# Autodesk Inventor assembly: Basic Chassis
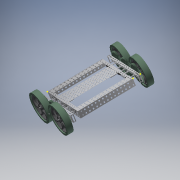
[picture p0: Inventor's stored thumbnail of the model, 180x180]
Saved by Autodesk Inventor 2018 (Build 220112000, 112)
## iProperties
Created: 2018-10-17
Part Number: Basic Chassis
Document SubType Name: Assembly
Designer: USER
Author: USER
## Documents named in this file (9)
- C:\Users\USER\Downloads\Inventor\Basic Chassis.iam
- C:\Users\USER\Downloads\Inventor\flat metal frame.ipt
- C:\Users\USER\Downloads\Inventor\Wheel.ipt
- C:\Users\USER\Downloads\Inventor\2sqr x 2sqr metal frame.ipt
- C:\Users\USER\Downloads\Inventor\1sqr x 2sqr metal frame.ipt
- C:\Users\USER\Downloads\Inventor\Axle.ipt
- C:\Users\USER\Downloads\Inventor\Gear.ipt
- C:\Users\USER\Downloads\Inventor\Plastic Fastener.ipt
- C:\Users\USER\Downloads\Inventor\Metal Fastener.ipt
## Components (34 placed, 8 different names)
1. flat metal frame:1 — Rigid:6
2. Wheel:2
3. 2sqr x 2sqr metal frame:1 — Mate:1, Mate:2, Mate:3, Mate:4, Flush:2, Flush:5
4. 2sqr x 2sqr metal frame:2 — Mate:5, Mate:6
5. 1sqr x 2sqr metal frame:1 — Mate:1, Mate:2, Mate:5, Mate:6, Flush:1, Flush:6, Rigid:6, Rigid:7, Rigid:9, Rigid:11
6. 1sqr x 2sqr metal frame:2 — Mate:3, Mate:4, Flush:3, Flush:4, Rigid:15, Rigid:16, Rigid:17
7. 1sqr x 2sqr metal frame:3 — Flush:3, Flush:4, Flush:5, Rigid:23, Rigid:24
8. 1sqr x 2sqr metal frame:4 — Flush:1, Flush:2, Flush:6, Rigid:25, Rigid:26
9. Axle:1 — Rotational:1, Rigid:8, Rigid:14
10. Axle:7 — Rotational:2, Rigid:10
11. Gear:3 — Rigid:10, Rotation:1, Rotation:2
12. Gear:6 — Rigid:8, Rotation:1
13. Plastic Fastener:2 — Rigid:7, Rotational:1
14. Plastic Fastener:6 — Rigid:9, Rotational:2
15. Plastic Fastener:7 — Rigid:11, Rotational:3
16. Axle:8 — Rotational:3, Rigid:12, Rigid:13
17. Gear:7 — Rigid:12, Rotation:2
18. Wheel:3 — Rigid:13
19. Wheel:4 — Rigid:14
20. Plastic Fastener:8 — Rigid:15, Rotational:4
21. Plastic Fastener:9 — Rigid:16, Rotational:5
22. Plastic Fastener:10 — Rigid:17, Rotational:6
23. Axle:9 — Rotational:6, Rigid:18, Rigid:22
24. Axle:10 — Rotational:4, Rigid:20, Rigid:21
25. Axle:11 — Rotational:5, Rigid:19
26. Gear:8 — Rigid:19, Rotation:3, Rotation:4
27. Gear:9 — Rigid:18, Rotation:3
28. Gear:10 — Rigid:20, Rotation:4
29. Wheel:5 — Rigid:21
30. Wheel:6 — Rigid:22
31. Metal Fastener:1 — Rigid:23
32. Metal Fastener:2 — Rigid:25
33. Metal Fastener:3 — Rigid:24
34. Metal Fastener:4 — Rigid:26
## Relationships (43: WeldJoint 21, Mate 6, Flush 6, RevoluteJoint 6, RelateRotation 4)
- Mate:1: 2sqr x 2sqr metal frame:1 ↔ 1sqr x 2sqr metal frame:1
- Mate:2: 2sqr x 2sqr metal frame:1 ↔ 1sqr x 2sqr metal frame:1
- Mate:3: 2sqr x 2sqr metal frame:1 ↔ 1sqr x 2sqr metal frame:2
- Mate:4: 2sqr x 2sqr metal frame:1 ↔ 1sqr x 2sqr metal frame:2
- Mate:5: 2sqr x 2sqr metal frame:2 ↔ 1sqr x 2sqr metal frame:1
- Mate:6: 2sqr x 2sqr metal frame:2 ↔ 1sqr x 2sqr metal frame:1
- Flush:1 (-25.4 mm): 1sqr x 2sqr metal frame:1 ↔ 1sqr x 2sqr metal frame:4
- Flush:2: 2sqr x 2sqr metal frame:1 ↔ 1sqr x 2sqr metal frame:4
- Flush:3 (-25.4 mm): 1sqr x 2sqr metal frame:2 ↔ 1sqr x 2sqr metal frame:3
- Flush:4: 1sqr x 2sqr metal frame:2 ↔ 1sqr x 2sqr metal frame:3
- Flush:5: 2sqr x 2sqr metal frame:1 ↔ 1sqr x 2sqr metal frame:3
- Flush:6: 1sqr x 2sqr metal frame:1 ↔ 1sqr x 2sqr metal frame:4
- Rigid:6 [WeldJoint]: flat metal frame:1 ↔ 1sqr x 2sqr metal frame:1
- Rigid:7 [WeldJoint]: 1sqr x 2sqr metal frame:1 ↔ Plastic Fastener:2
- Rotational:1 [RevoluteJoint] (-25 mm): Axle:1 ↔ Plastic Fastener:2
- Rigid:8 [WeldJoint] (-20 mm): Axle:1 ↔ Gear:6
- Rigid:9 [WeldJoint]: 1sqr x 2sqr metal frame:1 ↔ Plastic Fastener:6
- Rotational:2 [RevoluteJoint] (-25 mm): Axle:7 ↔ Plastic Fastener:6
- Rigid:10 [WeldJoint] (-20 mm): Axle:7 ↔ Gear:3
- Rotation:1 [RelateRotation] (1 ul): Gear:3 ↔ Gear:6
- Rigid:11 [WeldJoint]: 1sqr x 2sqr metal frame:1 ↔ Plastic Fastener:7
- Rotational:3 [RevoluteJoint] (-25 mm): Plastic Fastener:7 ↔ Axle:8
- Rigid:12 [WeldJoint] (-20 mm): Axle:8 ↔ Gear:7
- Rotation:2 [RelateRotation] (1 ul): Gear:3 ↔ Gear:7
- Rigid:13 [WeldJoint] (-15 mm): Axle:8 ↔ Wheel:3
- Rigid:14 [WeldJoint] (-15 mm): Axle:1 ↔ Wheel:4
- Rigid:15 [WeldJoint]: 1sqr x 2sqr metal frame:2 ↔ Plastic Fastener:8
- Rigid:16 [WeldJoint]: 1sqr x 2sqr metal frame:2 ↔ Plastic Fastener:9
- Rigid:17 [WeldJoint]: 1sqr x 2sqr metal frame:2 ↔ Plastic Fastener:10
- Rotational:4 [RevoluteJoint] (25 mm): Plastic Fastener:8 ↔ Axle:10
- Rotational:5 [RevoluteJoint] (-25 mm): Plastic Fastener:9 ↔ Axle:11
- Rotational:6 [RevoluteJoint] (-25 mm): Plastic Fastener:10 ↔ Axle:9
- Rigid:18 [WeldJoint] (-20 mm): Axle:9 ↔ Gear:9
- Rigid:19 [WeldJoint] (-22 mm): Axle:11 ↔ Gear:8
- Rotation:3 [RelateRotation] (1 ul): Gear:8 ↔ Gear:9
- Rigid:20 [WeldJoint] (-20 mm): Axle:10 ↔ Gear:10
- Rotation:4 [RelateRotation] (1 ul): Gear:8 ↔ Gear:10
- Rigid:21 [WeldJoint] (-15 mm): Axle:10 ↔ Wheel:5
- Rigid:22 [WeldJoint] (-15 mm): Axle:9 ↔ Wheel:6
- Rigid:23 [WeldJoint]: 1sqr x 2sqr metal frame:3 ↔ Metal Fastener:1
- Rigid:24 [WeldJoint]: 1sqr x 2sqr metal frame:3 ↔ Metal Fastener:3
- Rigid:25 [WeldJoint]: 1sqr x 2sqr metal frame:4 ↔ Metal Fastener:2
- Rigid:26 [WeldJoint]: 1sqr x 2sqr metal frame:4 ↔ Metal Fastener:4
